# Autodesk Inventor assembly: 1 Piece Support Assembly
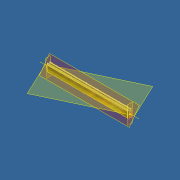
[picture p0: Inventor's stored thumbnail of the model, 180x180]
Saved by Autodesk Inventor 2011 SP1 (Build 150282100, 282)
## iProperties
Created: 2006-06-01
Part Number: 1 Piece Support Assembly
Document SubType Name: Assembly
Designer: Jon
Author: Jon
## Documents named in this file (4)
- C:\Documents and Settings\jdyne\My Documents\Inventor\EDM Beamline 2010\EDM Beamline\Field plates v3\1 Piece Support Assembly.iam
- C:\Documents and Settings\jdyne\My Documents\Inventor\EDM Beamline 2010\EDM Beamline\Field plates v3\1 Piece Support Plate.ipt
- C:\Documents and Settings\jdyne\My Documents\Inventor\EDM Beamline 2010\EDM Beamline\Field plates\Long rod.ipt
- C:\Documents and Settings\jdyne\My Documents\Inventor\EDM Beamline 2010\EDM Beamline\Field plates v3\Field Plate & Rods.iam
## Components (8 placed, 3 different names)
1. 1 Piece Support Plate:1 — Mate:1, Mate:2, Mate:3, Mate:4, Insert:1, Insert:4
2. Field Plate & Rods:1 [sub-assembly] — Mate:3, Mate:4, Mate:5, Mate:6, Flush:1, Mate:7, Mate:9, Mate:10, Mate:12, Mate:15, Mate:16
3. Field Plate & Rods:2 [sub-assembly] — Mate:1, Mate:2, Flush:2, Angle:1, Mate:11, Mate:14
4. 1 Piece Support Plate:2 — Mate:5, Mate:6, Flush:1, Flush:2, Insert:2, Insert:3
5. Long rod:1 — Insert:1
6. Long rod:2 — Insert:2
7. Long rod:3 — Insert:3
8. Long rod:4 — Insert:4
## Relationships (24: Mate 17, Insert 4, Flush 2, Angle 1)
- Mate:1: 1 Piece Support Plate:1 ↔ Field Plate & Rods:2
- Mate:2: 1 Piece Support Plate:1 ↔ Field Plate & Rods:2
- Mate:3: 1 Piece Support Plate:1 ↔ Field Plate & Rods:1
- Mate:4: 1 Piece Support Plate:1 ↔ Field Plate & Rods:1
- Mate:5: Field Plate & Rods:1 ↔ 1 Piece Support Plate:2
- Mate:6: Field Plate & Rods:1 ↔ 1 Piece Support Plate:2
- Flush:1 (-10 mm): Field Plate & Rods:1 ↔ 1 Piece Support Plate:2
- Flush:2 (-10 mm): Field Plate & Rods:2 ↔ 1 Piece Support Plate:2
- Insert:1: 1 Piece Support Plate:1 ↔ Long rod:1
- Insert:2: 1 Piece Support Plate:2 ↔ Long rod:2
- Insert:3: 1 Piece Support Plate:2 ↔ Long rod:3
- Insert:4: 1 Piece Support Plate:1 ↔ Long rod:4
- Mate:7: Field Plate & Rods:1
- Angle:1 (90 deg): Field Plate & Rods:2
- Mate:8
- Mate:9: Field Plate & Rods:1
- Mate:10: Field Plate & Rods:1
- Mate:11: Field Plate & Rods:2
- Mate:12: Field Plate & Rods:1
- Mate:13
- Mate:14: Field Plate & Rods:2
- Mate:15: Field Plate & Rods:1
- Mate:16: Field Plate & Rods:1
- Mate:17
